# Autodesk Inventor assembly: DribblerUnit
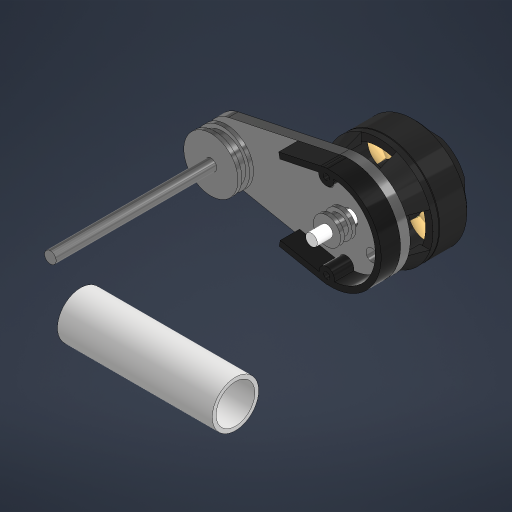
[picture p0: Inventor's stored thumbnail of the model, 512x512]
Saved by Autodesk Inventor 2024.2 (Build 282272000, 272)
## iProperties
Created: 2023-12-22
Part Number: DribblerUnit
Document SubType Name: Assembly
Designer: Hanaoka
Author: Hanaoka
## Documents named in this file (9)
- G:\共有ドライブ\reRo\05_個人\hanaoka\inventor\DribblerUnit.iam
- G:\共有ドライブ\reRo\05_個人\hanaoka\inventor\SilliconeTube_Dribbler.ipt
- G:\共有ドライブ\reRo\05_個人\hanaoka\inventor\C2822_BLDC\C2822_BLDC.ipt
- G:\共有ドライブ\reRo\05_個人\hanaoka\inventor\Dribler_main.ipt
- G:\共有ドライブ\reRo\05_個人\hanaoka\inventor\Misumi\Bearing_C-FL673ZZ\Bearing_C-FL673ZZ.ipt
- G:\共有ドライブ\reRo\05_個人\hanaoka\inventor\Shaft_3x50.ipt
- G:\共有ドライブ\reRo\05_個人\hanaoka\inventor\Pulley_MotorSide.ipt
- G:\共有ドライブ\reRo\05_個人\hanaoka\inventor\Pulley_OutSide.ipt
- G:\共有ドライブ\reRo\05_個人\hanaoka\inventor\MotorCover.ipt
## Components (8 placed, 8 different names)
1. SilliconeTube_Dribbler:1
2. C2822_BLDC:1 — フラッシュ:1, 挿入:3
3. Dribler_main:1 — フラッシュ:1, 挿入:1, フラッシュ:2, フラッシュ:3
4. Bearing_C-FL673ZZ:1 — 挿入:1, 挿入:2
5. Shaft_3x50:1 — 挿入:2, 挿入:4
6. Pulley_MotorSide:1 — 挿入:3
7. Pulley_OutSide:1 — 挿入:4
8. MotorCover:1 — フラッシュ:2, フラッシュ:3
## Relationships (7: Insert 4, Flush 3)
- フラッシュ:1 [Flush]: C2822_BLDC:1 ↔ Dribler_main:1
- 挿入:1 [Insert]: Dribler_main:1 ↔ Bearing_C-FL673ZZ:1
- 挿入:2 [Insert]: Bearing_C-FL673ZZ:1 ↔ Shaft_3x50:1
- 挿入:3 [Insert] (4 mm): C2822_BLDC:1 ↔ Pulley_MotorSide:1
- 挿入:4 [Insert] (4.5 mm): Shaft_3x50:1 ↔ Pulley_OutSide:1
- フラッシュ:2 [Flush]: Dribler_main:1 ↔ MotorCover:1
- フラッシュ:3 [Flush]: Dribler_main:1 ↔ MotorCover:1
